# Autodesk Inventor assembly: 베어링받침대결합
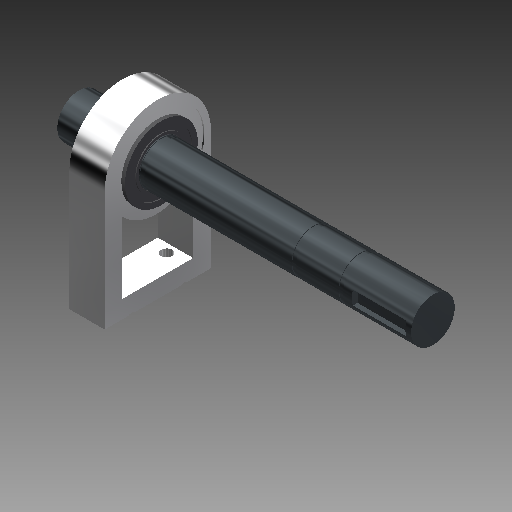
[picture p0: Inventor's stored thumbnail of the model, 512x512]
Saved by Autodesk Inventor 2017 (Build 210142000, 142)
## iProperties
Part Number: 베어링받침대결합
Material: 일반
Document SubType Name: Assembly
Designer: minom
Author: minom
## Documents named in this file (4)
- C:\Users\Minos\Documents\Inventor\Projects\2017 IRC Sumo Mino ver.2\베어링받침대결합.iam
- C:\Users\Minos\Documents\Inventor\Projects\2017 IRC Sumo Mino ver.2\베어링받침대.ipt
- C:\Users\Minos\Documents\Inventor\Projects\2017 IRC Sumo Mino ver.2\FL6700ZZ.ipt
- C:\Users\Minos\Documents\Inventor\Projects\2017 IRC Sumo Mino ver.2\10PI축.ipt
## Components (4 placed, 3 different names)
1. 베어링받침대:1 — 메이트:1, 메이트:2, 메이트:3, 메이트:4
2. FL6700ZZ:1 — 메이트:1, 메이트:2, 메이트:5
3. FL6700ZZ:2 — 메이트:3, 메이트:4, 플러쉬:1
4. 10PI축:1 — 메이트:5, 플러쉬:1
## Relationships (6: Mate 5, Flush 1)
- 메이트:1 [Mate]: 베어링받침대:1 ↔ FL6700ZZ:1
- 메이트:2 [Mate]: 베어링받침대:1 ↔ FL6700ZZ:1
- 메이트:3 [Mate]: 베어링받침대:1 ↔ FL6700ZZ:2
- 메이트:4 [Mate]: 베어링받침대:1 ↔ FL6700ZZ:2
- 메이트:5 [Mate]: FL6700ZZ:1 ↔ 10PI축:1
- 플러쉬:1 [Flush] (-9 mm): FL6700ZZ:2 ↔ 10PI축:1
